# Autodesk Inventor assembly: segment0
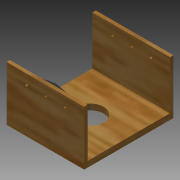
[picture p0: Inventor's stored thumbnail of the model, 180x180]
Saved by Autodesk Inventor 2013 (Build 170138000, 138)
## iProperties
Created: 2014-10-10
Part Number: segment0
Document SubType Name: Assembly
Designer: Masta
Author: Masta
## Documents named in this file (4)
- D:\DrOctopus\3D model\segment0.iam
- D:\DrOctopus\3D model\servo arm TGY-S8166M double.ipt
- D:\DrOctopus\3D model\segment0a.ipt
- D:\DrOctopus\3D model\segment0b.ipt
## Components (4 placed, 3 different names)
1. servo arm TGY-S8166M double:1 — Insert:1, Insert:2
2. segment0a:1 — Mate:1, Flush:2, Flush:3, Insert:1, Insert:2
3. segment0a:2 — Mate:2, Flush:4, Flush:5
4. segment0b:1 — Mate:1, Flush:2, Flush:3, Mate:2, Flush:4, Flush:5
## Relationships (8: Flush 4, Mate 2, Insert 2)
- Mate:1: segment0a:1 ↔ segment0b:1
- Flush:2: segment0a:1 ↔ segment0b:1
- Flush:3: segment0a:1 ↔ segment0b:1
- Mate:2: segment0a:2 ↔ segment0b:1
- Flush:4: segment0a:2 ↔ segment0b:1
- Flush:5: segment0a:2 ↔ segment0b:1
- Insert:1: servo arm TGY-S8166M double:1 ↔ segment0a:1
- Insert:2: servo arm TGY-S8166M double:1 ↔ segment0a:1
